# Autodesk Inventor assembly: Weird Spatula of lifting
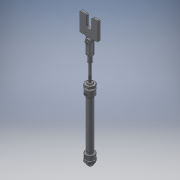
[picture p0: Inventor's stored thumbnail of the model, 180x180]
Saved by Autodesk Inventor 2018 (Build 220112000, 112)
## iProperties
Created: 2019-01-21
Part Number: Weird Spatula of lifting
Document SubType Name: Assembly
Designer: maste
Author: maste
## Documents named in this file (5)
- C:\Users\maste\OneDrive\Documents\GitHub\2019CAD\Drivebase but Calvin is a mad man\Weird Spatula of lifting.iam
- C:\Users\maste\OneDrive\Documents\GitHub\2019CAD\Drivebase but Calvin is a mad man\6071K110_FORGED CLEVIS ROD END.ipt
- C:\Users\maste\OneDrive\Documents\GitHub\2019CAD\Drivebase but Calvin is a mad man\6498K008_ROUND BODY AIR CYLINDER.ipt
- C:\Users\maste\OneDrive\Documents\GitHub\2019CAD\Drivebase but Calvin is a mad man\97235K174_TYPE 18-8 STAINLESS STEEL SLOTTED SHIM W  TAB.ipt
- C:\Users\maste\OneDrive\Documents\GitHub\2019CAD\Drivebase but Calvin is a mad man\97235K612_TYPE 18-8 STAINLESS STEEL SLOTTED SHIM W  TAB.ipt
## Components (4 placed, 4 different names)
1. 6071K110_FORGED CLEVIS ROD END:1 — Mate:2, Mate:3, Angle:1, Mate:4, Flush:3
2. 6498K008_ROUND BODY AIR CYLINDER:1 — Mate:4, Flush:3
3. 97235K174_TYPE 18-8 STAINLESS STEEL SLOTTED SHIM W  TAB:1 — Mate:1, Flush:1, Flush:2, Angle:1
4. 97235K612_TYPE 18-8 STAINLESS STEEL SLOTTED SHIM W  TAB:1 — Mate:1, Flush:1, Flush:2, Mate:2, Mate:3
## Relationships (8: Mate 4, Flush 3, Angle 1)
- Mate:1: 97235K174_TYPE 18-8 STAINLESS STEEL SLOTTED SHIM W  TAB:1 ↔ 97235K612_TYPE 18-8 STAINLESS STEEL SLOTTED SHIM W  TAB:1
- Flush:1: 97235K174_TYPE 18-8 STAINLESS STEEL SLOTTED SHIM W  TAB:1 ↔ 97235K612_TYPE 18-8 STAINLESS STEEL SLOTTED SHIM W  TAB:1
- Flush:2: 97235K174_TYPE 18-8 STAINLESS STEEL SLOTTED SHIM W  TAB:1 ↔ 97235K612_TYPE 18-8 STAINLESS STEEL SLOTTED SHIM W  TAB:1
- Mate:2: 6071K110_FORGED CLEVIS ROD END:1 ↔ 97235K612_TYPE 18-8 STAINLESS STEEL SLOTTED SHIM W  TAB:1
- Mate:3: 6071K110_FORGED CLEVIS ROD END:1 ↔ 97235K612_TYPE 18-8 STAINLESS STEEL SLOTTED SHIM W  TAB:1
- Angle:1 (180 deg): 6071K110_FORGED CLEVIS ROD END:1 ↔ 97235K174_TYPE 18-8 STAINLESS STEEL SLOTTED SHIM W  TAB:1
- Mate:4: 6071K110_FORGED CLEVIS ROD END:1 ↔ 6498K008_ROUND BODY AIR CYLINDER:1
- Flush:3: 6071K110_FORGED CLEVIS ROD END:1 ↔ 6498K008_ROUND BODY AIR CYLINDER:1
